# Autodesk Inventor assembly: Rear Panel Assembly
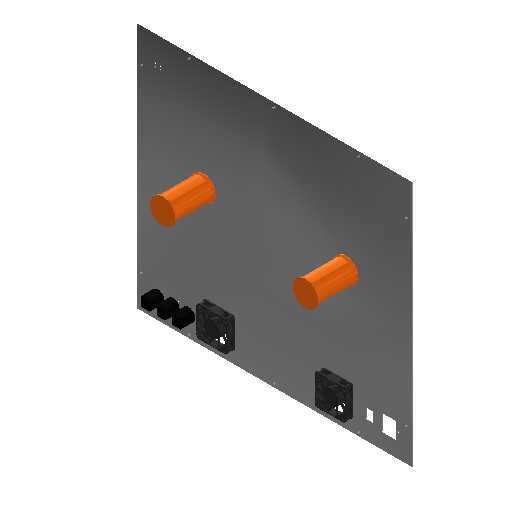
[picture p0: Inventor's stored thumbnail of the model, 512x512]
Saved by Autodesk Inventor 2023.2 (Build 272271000, 271)
## iProperties
Created: 2023-02-06
Part Number: Rear Panel Assembly
Document SubType Name: Assembly
Designer: remop
Author: remop
## Documents named in this file (6)
- C:\Users\remop\OneDrive\Documents\Inventor\3D Printers\LuEVO\Mk5_FullKinematic\Frame and Panels\Rear Panel Assembly.iam
- C:\Users\remop\OneDrive\Documents\Inventor\3D Printers\LuEVO\Mk5_FullKinematic\Frame and Panels\Rear Panel.ipt
- C:\Users\remop\OneDrive\Documents\Inventor\Content Center Files\R2023\en-US\AS 1420\AS 1420 - 1973 - M3 x 6.ipt
- C:\Users\remop\OneDrive\Documents\Inventor\3D Printers\LuEVO\Mk5_FullKinematic\Electronics\60mm x 15mm DC Fan v9\60mm x 15mm DC Fan v9.iam
- C:\Users\remop\OneDrive\Documents\Inventor\3D Printers\LuEVO\Mk5_FullKinematic\Electronics\Delock Panel Connector.ipt
- C:\Users\remop\OneDrive\Documents\Inventor\3D Printers\LuEVO\Mk5_FullKinematic\Filament Spool Holder.ipt
## Components (18 placed, 5 different names)
1. Rear Panel:1 — Insert:1, Insert:2, Insert:3, Insert:4, Insert:5, Insert:6, Insert:7, Insert:8, Insert:9, Insert:10, Rigid:1, Rigid:2, Rigid:3, Rigid:4, Rigid:5, Rigid:6, Rigid:7
2. AS 1420 - Metric M3 x 6:1 — Insert:1
3. AS 1420 - Metric M3 x 6:2 — Insert:2
4. AS 1420 - Metric M3 x 6:3 — Insert:3
5. AS 1420 - Metric M3 x 6:4 — Insert:4
6. AS 1420 - Metric M3 x 6:5 — Insert:5
7. AS 1420 - Metric M3 x 6:6 — Insert:6
8. AS 1420 - Metric M3 x 6:7 — Insert:7
9. AS 1420 - Metric M3 x 6:8 — Insert:8
10. AS 1420 - Metric M3 x 6:9 — Insert:9
11. AS 1420 - Metric M3 x 6:10 — Insert:10
12. 60mm x 15mm DC Fan v9:1 [sub-assembly] — Rigid:2
13. 60mm x 15mm DC Fan v9:2 [sub-assembly] — Rigid:1
14. Delock Panel Connector:1 — Rigid:5
15. Delock Panel Connector:2 — Rigid:4
16. Delock Panel Connector:3 — Rigid:3
17. Filament Spool Holder:1 — Rigid:6
18. Filament Spool Holder:2 — Rigid:7
## Relationships (17: Insert 10, WeldJoint 7)
- Insert:1: Rear Panel:1 ↔ AS 1420 - Metric M3 x 6:1
- Insert:2: Rear Panel:1 ↔ AS 1420 - Metric M3 x 6:2
- Insert:3: Rear Panel:1 ↔ AS 1420 - Metric M3 x 6:3
- Insert:4: Rear Panel:1 ↔ AS 1420 - Metric M3 x 6:4
- Insert:5: Rear Panel:1 ↔ AS 1420 - Metric M3 x 6:5
- Insert:6: Rear Panel:1 ↔ AS 1420 - Metric M3 x 6:6
- Insert:7: Rear Panel:1 ↔ AS 1420 - Metric M3 x 6:7
- Insert:8: Rear Panel:1 ↔ AS 1420 - Metric M3 x 6:8
- Insert:9: Rear Panel:1 ↔ AS 1420 - Metric M3 x 6:9
- Insert:10: Rear Panel:1 ↔ AS 1420 - Metric M3 x 6:10
- Rigid:1 [WeldJoint]: Rear Panel:1 ↔ 60mm x 15mm DC Fan v9:2
- Rigid:2 [WeldJoint]: Rear Panel:1 ↔ 60mm x 15mm DC Fan v9:1
- Rigid:3 [WeldJoint]: Rear Panel:1 ↔ Delock Panel Connector:3
- Rigid:4 [WeldJoint]: Rear Panel:1 ↔ Delock Panel Connector:2
- Rigid:5 [WeldJoint]: Rear Panel:1 ↔ Delock Panel Connector:1
- Rigid:6 [WeldJoint]: Rear Panel:1 ↔ Filament Spool Holder:1
- Rigid:7 [WeldJoint]: Rear Panel:1 ↔ Filament Spool Holder:2
